# Autodesk Inventor assembly: Ensamble
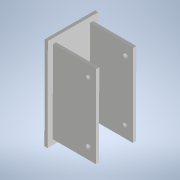
[picture p0: Inventor's stored thumbnail of the model, 180x180]
Saved by Autodesk Inventor 2022 (Build 260153000, 153)
## iProperties
Created: 2021-10-21
Part Number: Ensamble
Document SubType Name: Assembly
Designer: Administrador
Author: Administrador
## Documents named in this file (4)
- C:\Users\Administrador\Desktop\Octavo Semestre\Robótica Industrial\Robot\Base Camara\Ensamble.iam
- C:\Users\Administrador\Desktop\Octavo Semestre\Robótica Industrial\Robot\Cuerpo\PartesCuerpo\Estella Servo1.ipt
- C:\Users\Administrador\Desktop\Octavo Semestre\Robótica Industrial\Robot\Base Camara\Part1.ipt
- C:\Users\Administrador\Desktop\Octavo Semestre\Robótica Industrial\Robot\Base Camara\Part2.ipt
## Components (4 placed, 3 different names)
1. Estella Servo1:1 — Flush:1, Flush:2
2. Part1:1 — Flush:2, Flush:4, Mate:6, Mate:7, Mate:8, Flush:5, Mate:9
3. Part2:1 — Flush:4, Mate:6, Mate:7
4. Part2:2 — Mate:8, Flush:5, Mate:9
## Relationships (8: Flush 4, Mate 4)
- Flush:1: Estella Servo1:1
- Flush:2: Estella Servo1:1 ↔ Part1:1
- Flush:4: Part1:1 ↔ Part2:1
- Mate:6: Part1:1 ↔ Part2:1
- Mate:7: Part1:1 ↔ Part2:1
- Mate:8: Part1:1 ↔ Part2:2
- Flush:5: Part1:1 ↔ Part2:2
- Mate:9: Part1:1 ↔ Part2:2
